# Autodesk Inventor assembly: Synchronous Belts Transmission1_MIR
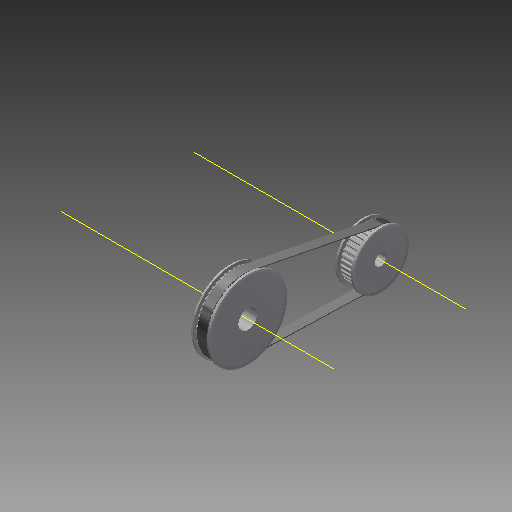
[picture p0: Inventor's stored thumbnail of the model, 512x512]
Saved by Autodesk Inventor 2019.4 (Build 234330000, 330)
## iProperties
Created: 2019-11-02
Part Number: Synchronous Belts Transmission1_MIR
Document SubType Name: Assembly
Designer: Mark
Mass: 953.385 g
Surface Area: 418.584 cm^2
Volume: 125.858 cm^3
Density: 7.57509 g/cm^3
Author: admin
## Documents named in this file (4)
- C:\Users\admin\Desktop\FRC 2020 Engineering\GitHub\7738-CAD-prep\Butterfly Drive Mk2\Butterfly Module\Butterfly Drive Module\Design Accelerator\Synchronous Belts Transmission1_MIR.iam
- C:\Users\admin\Desktop\FRC 2020 Engineering\GitHub\7738-CAD-prep\Butterfly Drive Mk2\Butterfly Module\Butterfly Drive Module\Design Accelerator\Synchronous Belt1_MIR.ipt
- C:\Users\admin\Desktop\FRC 2020 Engineering\GitHub\7738-CAD-prep\Butterfly Drive Mk2\Butterfly Module\Butterfly Drive Module\Design Accelerator\Synchronous Pulley11_MIR.ipt
- C:\Users\admin\Desktop\FRC 2020 Engineering\GitHub\7738-CAD-prep\Butterfly Drive Mk2\Butterfly Module\Butterfly Drive Module\Design Accelerator\Synchronous Pulley21_MIR.ipt
## Components (3 placed, 3 different names)
1. Synchronous Belt1_MIR:1 — Mate:2, Mate:1, Flush:1, Mate:4, Mate:3, Flush:2
2. Synchronous Pulley11_MIR:1 — Mate:2, Mate:1, Flush:1, Rotation:1
3. Synchronous Pulley21_MIR:1 — Mate:4, Mate:3, Flush:2, Rotation:1
## Relationships (7: Flush 4, Mate 2, RelateRotation 1)
- Mate:2 [Flush]: Synchronous Belt1_MIR:1 ↔ Synchronous Pulley11_MIR:1
- Mate:1: Synchronous Belt1_MIR:1 ↔ Synchronous Pulley11_MIR:1
- Flush:1: Synchronous Belt1_MIR:1 ↔ Synchronous Pulley11_MIR:1
- Mate:4 [Flush]: Synchronous Belt1_MIR:1 ↔ Synchronous Pulley21_MIR:1
- Mate:3: Synchronous Belt1_MIR:1 ↔ Synchronous Pulley21_MIR:1
- Flush:2: Synchronous Belt1_MIR:1 ↔ Synchronous Pulley21_MIR:1
- Rotation:1 [RelateRotation] (1.4286 ul): Synchronous Pulley11_MIR:1 ↔ Synchronous Pulley21_MIR:1
